# Autodesk Inventor assembly: Slope_LowEndHi-FM
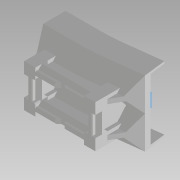
[picture p0: Inventor's stored thumbnail of the model, 180x180]
Saved by Autodesk Inventor 2021 (Build 250183000, 183)
## iProperties
Created: 2021-03-16
Part Number: Slope_LowEndHi-FM
Document SubType Name: Assembly
Designer: kumagai
Author: kumagai
## Documents named in this file (8)
- X:\Develop\CAD\PlaRails\VPUSlope\Slope_LowEndHi.iam
- X:\Develop\CAD\PlaRails\VPUSlope\Slope_LowEndHi.ipt
- X:\Develop\CAD\PlaRails\ViaductPillarUnit\VPU_EdgeBottom.ipt
- X:\Develop\CAD\PlaRails\GlobalParameter.ipt
- X:\Develop\CAD\PlaRails\RailJointFemale_filled.ipt
- X:\Develop\CAD\PlaRails\RailJointMale_filled.ipt
- Slope_LowEndHi-FM.iam
- Slope_LowEndHi-MM.iam
## Components (6 placed, 4 different names)
1. Slope_LowEndHi:1 — フラッシュ:3, メイト:2, メイト:3, メイト:4, メイト:5, メイト:6, フラッシュ:4, フラッシュ:5, メイト:7, メイト:8, メイト:9, フラッシュ:6
2. VPU_EdgeBottom:1 — メイト:1, フラッシュ:1, フラッシュ:2, フラッシュ:3, メイト:2, メイト:7
3. VPU_EdgeBottom:2 — メイト:1, フラッシュ:1, フラッシュ:2
4. RailJointFemale_filled:1 — メイト:4, メイト:5, フラッシュ:4
5. RailJointMale_filled:1 — メイト:3, メイト:6, フラッシュ:5
6. RailJointMale_filled:2 — メイト:8, メイト:9, フラッシュ:6
## Relationships (15: Mate 9, Flush 6)
- メイト:1 [Mate]: VPU_EdgeBottom:1 ↔ VPU_EdgeBottom:2
- フラッシュ:1 [Flush]: VPU_EdgeBottom:1 ↔ VPU_EdgeBottom:2
- フラッシュ:2 [Flush]: VPU_EdgeBottom:1 ↔ VPU_EdgeBottom:2
- フラッシュ:3 [Flush]: Slope_LowEndHi:1 ↔ VPU_EdgeBottom:1
- メイト:2 [Mate] (-33 mm): Slope_LowEndHi:1 ↔ VPU_EdgeBottom:1
- メイト:3 [Mate]: Slope_LowEndHi:1 ↔ RailJointMale_filled:1
- メイト:4 [Mate]: Slope_LowEndHi:1 ↔ RailJointFemale_filled:1
- メイト:5 [Mate]: Slope_LowEndHi:1 ↔ RailJointFemale_filled:1
- メイト:6 [Mate]: Slope_LowEndHi:1 ↔ RailJointMale_filled:1
- フラッシュ:4 [Flush]: Slope_LowEndHi:1 ↔ RailJointFemale_filled:1
- フラッシュ:5 [Flush]: Slope_LowEndHi:1 ↔ RailJointMale_filled:1
- メイト:7 [Mate] (-20 mm): Slope_LowEndHi:1 ↔ VPU_EdgeBottom:1
- メイト:8 [Mate]: Slope_LowEndHi:1 ↔ RailJointMale_filled:2
- メイト:9 [Mate]: Slope_LowEndHi:1 ↔ RailJointMale_filled:2
- フラッシュ:6 [Flush]: Slope_LowEndHi:1 ↔ RailJointMale_filled:2
## Named parameters: PrinterOffset = 0 mm, StraightLength = 215 mm, RailWidth = 38 mm, OuterWall = 2 mm, InnerWall = 2.4 mm, InsideWidth = 18.6 mm, RailHeight = 8.4 mm, RailDepth = 3.2 mm, ConnectorLength = 15 mm, JointMW1 = 13 mm, JointMW2 = 9.4 mm, JointMH = 9 mm, JointFW1 = 13.3 mm, JointFW2 = 9.6 mm, JointFH = 9.5 mm, DoubleWidth = 60 mm, ViaductHeight = 66 mm, SupportGap = 0.2 mm, SupportRib = 0.5 mm
